# Autodesk Inventor assembly: rev1 base short wall
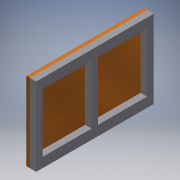
[picture p0: Inventor's stored thumbnail of the model, 180x180]
Saved by Autodesk Inventor 2017 (Build 210142000, 142)
## iProperties
Created: 2019-05-04
Part Number: rev1 base short wall
Document SubType Name: Assembly
Designer: Roman
Author: Roman
## Documents named in this file (4)
- C:\Users\Roman\Documents\CAD\enclosure rev1\rev2 base\rev1 small wall\rev1 base short wall.iam
- C:\Users\Roman\Documents\CAD\enclosure rev1\rev2 base\rev1 small wall\rev1 base short wall backplane.ipt
- C:\Users\Roman\Documents\CAD\enclosure rev1\rev2 base\rev1 small wall\rev1 base short wall h stud.ipt
- C:\Users\Roman\Documents\CAD\enclosure rev1\rev2 base\rev1 large wall\rev1 base large wall v stud.ipt
## Components (6 placed, 3 different names)
1. rev1 base short wall backplane:1 — Mate:1, Mate:2, Flush:1, Flush:2, Flush:3, Flush:4, Flush:5, Mate:4
2. rev1 base short wall h stud:1 — Mate:2, Flush:1, Flush:3
3. rev1 base short wall h stud:2 — Mate:1, Flush:2, Flush:4, Mate:3
4. rev1 base large wall v stud:1 — Mate:3, Flush:5, Mate:4
5. rev1 base large wall v stud:2
6. rev1 base large wall v stud:3
## Component patterns: (3 elements, first: rev1 base large wall v stud:1)
## Relationships (9: Flush 5, Mate 4)
- Mate:1: rev1 base short wall backplane:1 ↔ rev1 base short wall h stud:2
- Mate:2: rev1 base short wall backplane:1 ↔ rev1 base short wall h stud:1
- Flush:1: rev1 base short wall backplane:1 ↔ rev1 base short wall h stud:1
- Flush:2: rev1 base short wall backplane:1 ↔ rev1 base short wall h stud:2
- Flush:3: rev1 base short wall backplane:1 ↔ rev1 base short wall h stud:1
- Flush:4: rev1 base short wall backplane:1 ↔ rev1 base short wall h stud:2
- Mate:3: rev1 base short wall h stud:2 ↔ rev1 base large wall v stud:1
- Flush:5: rev1 base short wall backplane:1 ↔ rev1 base large wall v stud:1
- Mate:4: rev1 base short wall backplane:1 ↔ rev1 base large wall v stud:1
